# Autodesk Inventor assembly: BaseAssembly
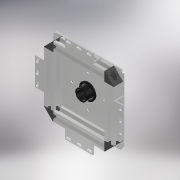
[picture p0: Inventor's stored thumbnail of the model, 180x180]
Saved by Autodesk Inventor 2020.3 (Build 243373000, 373)
## iProperties
Created: 2021-08-02
Part Number: BaseAssembly
Document SubType Name: Assembly
Designer: justi
Author: justi
## Documents named in this file (8)
- F:\UQ Engineering\2021 ~ 5th Year\Semester 2\METR4911-THESIS\FarmBot CAD\FarmBotV1\BaseAssembly.iam
- F:\UQ Engineering\2021 ~ 5th Year\Semester 2\METR4911-THESIS\FarmBot CAD\FarmBotV1\20x20x110mm.ipt
- F:\UQ Engineering\2021 ~ 5th Year\Semester 2\METR4911-THESIS\FarmBot CAD\FarmBotV1\VSlotHardware\Black Angle Corner Connector.ipt
- F:\UQ Engineering\2021 ~ 5th Year\Semester 2\METR4911-THESIS\FarmBot CAD\FarmBotV1\VSlotHardware\L bracket Custom.ipt
- F:\UQ Engineering\2021 ~ 5th Year\Semester 2\METR4911-THESIS\FarmBot CAD\FarmBotV1\BaseRotation\BaseTopPlate.ipt
- F:\UQ Engineering\2021 ~ 5th Year\Semester 2\METR4911-THESIS\FarmBot CAD\FarmBotV1\BaseRotation\ThrustBearingMount.ipt
- F:\UQ Engineering\2021 ~ 5th Year\Semester 2\METR4911-THESIS\FarmBot CAD\FarmBotV1\BaseRotation\ThrustBearing_OD_47_ID_25_W_15.ipt
- F:\UQ Engineering\2021 ~ 5th Year\Semester 2\METR4911-THESIS\FarmBot CAD\FarmBotV1\BaseRotation\BearingInsert.ipt
## Components (16 placed, 7 different names)
1. Black Angle Corner Connector:2 — Mate:29, Mate:30, Mate:35, Mate:36
2. Black Angle Corner Connector:4 — Mate:37, Mate:38
3. 20x20x110mm:3 — Mate:23, Flush:1, Flush:2, Mate:25
4. Black Angle Corner Connector:5 — Mate:27, Mate:28
5. Black Angle Corner Connector:6 — Mate:32, Mate:33
6. L bracket Custom:1 — Mate:23, Flush:1, Flush:2
7. 20x20x110mm:4 — Mate:27, Mate:28, Mate:29, Mate:30, Flush:9
8. L bracket Custom:2
9. 20x20x110mm:5 — Mate:32, Mate:33, Mate:37, Mate:39, Flush:11
10. L bracket Custom:3
11. 20x20x110mm:6 — Mate:35, Mate:36, Mate:38, Flush:10
12. L bracket Custom:4
13. BaseTopPlate:1 — Flush:10, Mate:39, Flush:11, Mate:40, Mate:41, Mate:42
14. ThrustBearingMount:1 — Mate:40, Mate:41, Mate:42, Mate:43, Mate:44
15. ThrustBearing_OD_47_ID_25_W_15:1 — Mate:43, Mate:44, Mate:45, Mate:46
16. BearingInsert:1 — Mate:45, Mate:46
## Relationships (38: Mate 27, Flush 11)
- [Mate]: 20x20x110mm:3 ↔ Black Angle Corner Connector:5
- [Mate]: 20x20x110mm:3 ↔ Black Angle Corner Connector:5
- [Mate]: 20x20x110mm:3 ↔ Black Angle Corner Connector:6
- [Mate]: 20x20x110mm:3 ↔ Black Angle Corner Connector:6
- Mate:23: 20x20x110mm:3 ↔ L bracket Custom:1
- Flush:1: 20x20x110mm:3 ↔ L bracket Custom:1
- Flush:2: 20x20x110mm:3 ↔ L bracket Custom:1
- Mate:25: 20x20x110mm:3
- [Mate]: 20x20x110mm:4 ↔ L bracket Custom:2
- [Flush]: 20x20x110mm:4 ↔ L bracket Custom:2
- [Flush]: 20x20x110mm:4 ↔ L bracket Custom:2
- Mate:27: Black Angle Corner Connector:5 ↔ 20x20x110mm:4
- Mate:28: Black Angle Corner Connector:5 ↔ 20x20x110mm:4
- Mate:29: Black Angle Corner Connector:2 ↔ 20x20x110mm:4
- Mate:30: Black Angle Corner Connector:2 ↔ 20x20x110mm:4
- [Mate]: 20x20x110mm:5 ↔ L bracket Custom:3
- [Flush]: 20x20x110mm:5 ↔ L bracket Custom:3
- [Flush]: 20x20x110mm:5 ↔ L bracket Custom:3
- Mate:32: Black Angle Corner Connector:6 ↔ 20x20x110mm:5
- Mate:33: Black Angle Corner Connector:6 ↔ 20x20x110mm:5
- [Mate]: 20x20x110mm:6 ↔ L bracket Custom:4
- [Flush]: 20x20x110mm:6 ↔ L bracket Custom:4
- [Flush]: 20x20x110mm:6 ↔ L bracket Custom:4
- Mate:35: Black Angle Corner Connector:2 ↔ 20x20x110mm:6
- Mate:36: Black Angle Corner Connector:2 ↔ 20x20x110mm:6
- Flush:9: 20x20x110mm:4
- Mate:37: Black Angle Corner Connector:4 ↔ 20x20x110mm:5
- Mate:38: Black Angle Corner Connector:4 ↔ 20x20x110mm:6
- Flush:10: 20x20x110mm:6 ↔ BaseTopPlate:1
- Mate:39: 20x20x110mm:5 ↔ BaseTopPlate:1
- Flush:11: 20x20x110mm:5 ↔ BaseTopPlate:1
- Mate:40: BaseTopPlate:1 ↔ ThrustBearingMount:1
- Mate:41: BaseTopPlate:1 ↔ ThrustBearingMount:1
- Mate:42: BaseTopPlate:1 ↔ ThrustBearingMount:1
- Mate:43: ThrustBearingMount:1 ↔ ThrustBearing_OD_47_ID_25_W_15:1
- Mate:44: ThrustBearingMount:1 ↔ ThrustBearing_OD_47_ID_25_W_15:1
- Mate:45: ThrustBearing_OD_47_ID_25_W_15:1 ↔ BearingInsert:1
- Mate:46: ThrustBearing_OD_47_ID_25_W_15:1 ↔ BearingInsert:1
## Named parameters: d32_d19 = 0 mm, d33_d22 = 0 mm, d34_d27 = 0 mm, d35_d29 = 0 mm, d51_d47 = 0 mm, d52_d48 = 0 mm, d53_d46 = 0 mm, d58_d47 = 0 mm, d59_d48 = 0 mm, d60_d46 = 0 mm, d63_d47 = 0 mm, d64_d48 = 0 mm, d65_d46 = 0 mm
